# Autodesk Inventor assembly: ARM PERHAPS use2
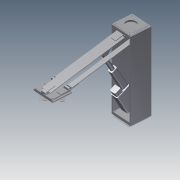
[picture p0: Inventor's stored thumbnail of the model, 180x180]
Saved by Autodesk Inventor 2011 (Build 150239000, 239)
## iProperties
Created: 2011-10-08
Part Number: ARM PERHAPS use2
Document SubType Name: Assembly
Designer: Matthew
Author: Matthew
## Documents named in this file (13)
- C:\Users\Matthew\Documents\matthew_autocad\prlite\arm perhaps\ARM PERHAPS use2.iam
- C:\Users\Matthew\Documents\matthew_autocad\prlite\arm perhaps\1.ipt
- C:\Users\Matthew\Documents\matthew_autocad\prlite\arm perhaps\2.ipt
- C:\Users\Matthew\Documents\matthew_autocad\prlite\arm perhaps\side.ipt
- C:\Users\Matthew\Documents\matthew_autocad\prlite\arm perhaps\back.ipt
- C:\Users\Matthew\Documents\matthew_autocad\prlite\arm perhaps\tb.ipt
- C:\Users\Matthew\Documents\matthew_autocad\prlite\arm perhaps\linac.iam
- C:\Users\Matthew\Documents\matthew_autocad\prlite\arm perhaps\linacconnect.ipt
- C:\Users\Matthew\Documents\matthew_autocad\prlite\arm perhaps\aluminum1.ipt
- C:\Users\Matthew\Documents\matthew_autocad\prlite\arm perhaps\linac arm1.ipt
- C:\Users\Matthew\Documents\matthew_autocad\prlite\arm perhaps\hinge.ipt
- C:\Users\Matthew\Documents\matthew_autocad\prlite\arm perhaps\aluminum2.ipt
- C:\Users\Matthew\Documents\matthew_autocad\prlite\arm perhaps\tb2.ipt
## Components (34 placed, 12 different names)
1. 2:1 — Mate:6, Mate:7, Flush:38
2. 1:1 — Mate:4, Mate:5, Mate:6, Mate:7, Mate:71
3. tb:1 — Mate:4, Mate:5, Mate:10, Mate:15, Mate:31, Flush:15, Flush:16, Mate:43, Flush:27, Mate:47, Mate:68, Mate:69, Mate:70, Mate:88
4. back:1 — Mate:10, Mate:11, Mate:44, Mate:49, Mate:62, Mate:77, Flush:44, Flush:46, Flush:47
5. linac:1 [sub-assembly] — Mate:13, Mate:14, Mate:27, Flush:12
6. aluminum1:1 — Mate:29, Flush:13, Mate:33, Mate:34, Flush:18, Flush:19, Flush:26, Mate:41, Mate:42
7. linac arm1:1 — Mate:27, Flush:12, Mate:30
8. linacconnect:1 — Mate:11, Mate:13, Mate:14, Mate:15, Mate:87
9. linacconnect:3 — Mate:29, Flush:13, Mate:30, Flush:19
10. tb:2 — Mate:56, Flush:32, Flush:33, Mate:57, Flush:34, Mate:58, Flush:35, Mate:79, Mate:80, Mate:81
11. hinge:1 — Mate:31, Flush:15, Flush:16, Flush:17, Mate:32
12. hinge:2 — Flush:17, Mate:32, Mate:33, Mate:34, Flush:18
13. hinge:4 — Mate:39, Flush:23, Mate:47, Mate:49
14. hinge:5 — Mate:39, Flush:23, Mate:50, Flush:29, Mate:51, Mate:89
15. hinge:6 — Mate:40, Flush:24, Mate:56, Flush:32, Flush:33
16. hinge:7 — Flush:20, Mate:35, Mate:43, Mate:44, Flush:27
17. hinge:8 — Mate:36, Flush:21, Mate:57, Flush:34
18. hinge:9 — Mate:36, Flush:21, Mate:52, Flush:30, Mate:53
19. hinge:10 — Flush:20, Mate:35, Mate:45, Mate:46, Flush:28
20. hinge:11 — Mate:37, Flush:22, Mate:54, Flush:31, Mate:55
21. hinge:12 — Mate:37, Flush:22, Mate:58, Flush:35
22. hinge:13 — Mate:40, Flush:24, Flush:26, Mate:41, Mate:42
23. aluminum2:1 — Mate:50, Flush:29, Mate:51, Mate:54, Flush:31, Mate:55
24. aluminum2:2 — Mate:45, Mate:46, Flush:28, Mate:52, Flush:30, Mate:53
25. tb:3 — Mate:62, Mate:64, Mate:65, Mate:72, Mate:73, Mate:74, Mate:78, Flush:42
26. 1:2 — Mate:64, Mate:65, Mate:66, Mate:67, Mate:75
27. 2:2 — Mate:66, Mate:67, Flush:38
28. tb2:1 — Mate:68, Mate:69, Mate:70, Mate:71, Mate:91, Mate:92, Flush:47
29. tb2:2 — Mate:72, Mate:73, Mate:74, Mate:75, Mate:90
30. side:1 — Mate:77, Mate:78, Mate:87, Flush:44, Mate:89, Mate:91
31. tb2:3 — Mate:79, Mate:80, Mate:81, Mate:84, Mate:85, Mate:86
32. 1:3 — Mate:82, Mate:83, Mate:84, Mate:85, Mate:86
33. 2:3 — Mate:82, Mate:83
34. side:2 — Flush:42, Mate:88, Flush:46, Mate:90, Mate:92
## Relationships (94: Mate 67, Flush 27)
- Mate:4: 1:1 ↔ tb:1
- Mate:5: 1:1 ↔ tb:1
- Mate:6: 2:1 ↔ 1:1
- Mate:7: 2:1 ↔ 1:1
- Mate:10: tb:1 ↔ back:1
- Mate:11: back:1 ↔ linacconnect:1
- Mate:13: linac:1 ↔ linacconnect:1
- Mate:14 (1.1049 mm): linac:1 ↔ linacconnect:1
- Mate:15 (365.76 mm): tb:1 ↔ linacconnect:1
- Mate:27: linac:1 ↔ linac arm1:1
- Flush:12: linac:1 ↔ linac arm1:1
- Mate:29: aluminum1:1 ↔ linacconnect:3
- Flush:13 (9.398 mm): aluminum1:1 ↔ linacconnect:3
- Mate:30: linac arm1:1 ↔ linacconnect:3
- Mate:31: tb:1 ↔ hinge:1
- Flush:15 (38.1 mm): tb:1 ↔ hinge:1
- Flush:16: tb:1 ↔ hinge:1
- Flush:17: hinge:1 ↔ hinge:2
- Mate:32: hinge:1 ↔ hinge:2
- Mate:33: aluminum1:1 ↔ hinge:2
- Mate:34: aluminum1:1 ↔ hinge:2
- Flush:18 (12.7 mm): aluminum1:1 ↔ hinge:2
- Flush:19 (69.85 mm): aluminum1:1 ↔ linacconnect:3
- Flush:20: hinge:7 ↔ hinge:10
- Mate:35: hinge:7 ↔ hinge:10
- Mate:36: hinge:8 ↔ hinge:9
- Flush:21: hinge:8 ↔ hinge:9
- Mate:37: hinge:11 ↔ hinge:12
- Flush:22: hinge:11 ↔ hinge:12
- Mate:39: hinge:4 ↔ hinge:5
- Flush:23: hinge:4 ↔ hinge:5
- Mate:40: hinge:6 ↔ hinge:13
- Flush:24: hinge:6 ↔ hinge:13
- Flush:26 (12.7 mm): aluminum1:1 ↔ hinge:13
- Mate:41: aluminum1:1 ↔ hinge:13
- Mate:42: aluminum1:1 ↔ hinge:13
- Mate:43: tb:1 ↔ hinge:7
- Mate:44: back:1 ↔ hinge:7
- Flush:27: tb:1 ↔ hinge:7
- Mate:45: hinge:10 ↔ aluminum2:2
- Mate:46: hinge:10 ↔ aluminum2:2
- Flush:28: hinge:10 ↔ aluminum2:2
- Mate:47: tb:1 ↔ hinge:4
- Mate:49: back:1 ↔ hinge:4
- Mate:50: hinge:5 ↔ aluminum2:1
- Flush:29: hinge:5 ↔ aluminum2:1
- Mate:51: hinge:5 ↔ aluminum2:1
- Mate:52: hinge:9 ↔ aluminum2:2
- Flush:30: hinge:9 ↔ aluminum2:2
- Mate:53: hinge:9 ↔ aluminum2:2
- Mate:54: hinge:11 ↔ aluminum2:1
- Flush:31: hinge:11 ↔ aluminum2:1
- Mate:55: hinge:11 ↔ aluminum2:1
- Mate:56: tb:2 ↔ hinge:6
- Flush:32: tb:2 ↔ hinge:6
- Flush:33 (38.1 mm): tb:2 ↔ hinge:6
- Mate:57: tb:2 ↔ hinge:8
- Flush:34: tb:2 ↔ hinge:8
- Mate:58: tb:2 ↔ hinge:12
- Flush:35: tb:2 ↔ hinge:12
- Mate:62: back:1 ↔ tb:3
- Mate:64: tb:3 ↔ 1:2
- Mate:65: tb:3 ↔ 1:2
- Mate:66: 1:2 ↔ 2:2
- Mate:67: 1:2 ↔ 2:2
- Flush:38: 2:1 ↔ 2:2
- Mate:68: tb:1 ↔ tb2:1
- Mate:69: tb:1 ↔ tb2:1
- Mate:70: tb:1 ↔ tb2:1
- Mate:71: 1:1 ↔ tb2:1
- Mate:72: tb:3 ↔ tb2:2
- Mate:73: tb:3 ↔ tb2:2
- Mate:74: tb:3 ↔ tb2:2
- Mate:75: 1:2 ↔ tb2:2
- Mate:77: back:1 ↔ side:1
- Mate:78: tb:3 ↔ side:1
- Mate:79: tb:2 ↔ tb2:3
- Mate:80: tb:2 ↔ tb2:3
- Mate:81: tb:2 ↔ tb2:3
- Mate:82: 1:3 ↔ 2:3
- Mate:83: 1:3 ↔ 2:3
- Mate:84: tb2:3 ↔ 1:3
- Mate:85: tb2:3 ↔ 1:3
- Mate:86: tb2:3 ↔ 1:3
- Mate:87 (34.798 mm): linacconnect:1 ↔ side:1
- Flush:42: tb:3 ↔ side:2
- Mate:88: tb:1 ↔ side:2
- Flush:44: back:1 ↔ side:1
- Flush:46: back:1 ↔ side:2
- Mate:89: hinge:5 ↔ side:1
- Mate:90: tb2:2 ↔ side:2
- Mate:91: tb2:1 ↔ side:1
- Mate:92: tb2:1 ↔ side:2
- Flush:47: back:1 ↔ tb2:1
